# Autodesk Inventor assembly: Electronics Endcap Starboard Assembly
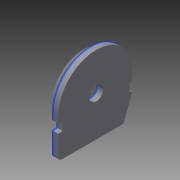
[picture p0: Inventor's stored thumbnail of the model, 180x180]
Saved by Autodesk Inventor 2015 (Build 190159000, 159)
## iProperties
Created: 2015-01-14
Part Number: Electronics Endcap Starboard Assembly
Document SubType Name: Assembly
Designer: Stackpole
Author: Stackpole
## Documents named in this file (6)
- C:\Users\Stackpole\Desktop\Brian G\V2.7\Electronics Tube\Electronics Endcaps\Electronics Endcap Starboard Assembly.iam
- C:\Users\Stackpole\Desktop\Brian G\V2.7\Electronics Tube\Electronics Endcaps\Electronics Endcaps Outer Gland Wall.ipt
- C:\Users\Stackpole\Desktop\Brian G\V2.7\Electronics Tube\Electronics Endcaps\Electronics Endcaps Inner Gland.ipt
- C:\Users\Stackpole\Desktop\Brian G\V2.7\Electronics Tube\Electronics Endcaps\Electronics Endcaps Inner Flange.ipt
- C:\Users\Stackpole\Desktop\Brian G\V2.7\Electronics Tube\Electronics Endcaps\Electronics Endcaps Middle Flange.ipt
- C:\Users\Stackpole\Desktop\Brian G\V2.7\Electronics Tube\Electronics Endcaps\Electronics Endcaps Outer Flange.ipt
## Components (5 placed, 5 different names)
1. Electronics Endcaps Outer Gland Wall:1 — Mate:1, Mate:2, Mate:3, Mate:5, Mate:9, Mate:11
2. Electronics Endcaps Inner Gland:1 — Mate:1, Mate:2, Mate:3, Mate:4, Mate:8
3. Electronics Endcaps Inner Flange:1 — Mate:4, Mate:5, Mate:6, Mate:7, Mate:8
4. Electronics Endcaps Middle Flange:1 — Mate:6, Mate:7, Mate:9, Mate:10, Flush:1
5. Electronics Endcaps Outer Flange:1 — Mate:10, Flush:1, Mate:11
## Relationships (12: Mate 11, Flush 1)
- Mate:1: Electronics Endcaps Outer Gland Wall:1 ↔ Electronics Endcaps Inner Gland:1
- Mate:2: Electronics Endcaps Outer Gland Wall:1 ↔ Electronics Endcaps Inner Gland:1
- Mate:3: Electronics Endcaps Outer Gland Wall:1 ↔ Electronics Endcaps Inner Gland:1
- Mate:4: Electronics Endcaps Inner Gland:1 ↔ Electronics Endcaps Inner Flange:1
- Mate:5: Electronics Endcaps Outer Gland Wall:1 ↔ Electronics Endcaps Inner Flange:1
- Mate:6: Electronics Endcaps Inner Flange:1 ↔ Electronics Endcaps Middle Flange:1
- Mate:7: Electronics Endcaps Inner Flange:1 ↔ Electronics Endcaps Middle Flange:1
- Mate:8: Electronics Endcaps Inner Gland:1 ↔ Electronics Endcaps Inner Flange:1
- Mate:9: Electronics Endcaps Outer Gland Wall:1 ↔ Electronics Endcaps Middle Flange:1
- Mate:10: Electronics Endcaps Middle Flange:1 ↔ Electronics Endcaps Outer Flange:1
- Flush:1: Electronics Endcaps Middle Flange:1 ↔ Electronics Endcaps Outer Flange:1
- Mate:11: Electronics Endcaps Outer Gland Wall:1 ↔ Electronics Endcaps Outer Flange:1
